# Autodesk Inventor assembly: robhand1
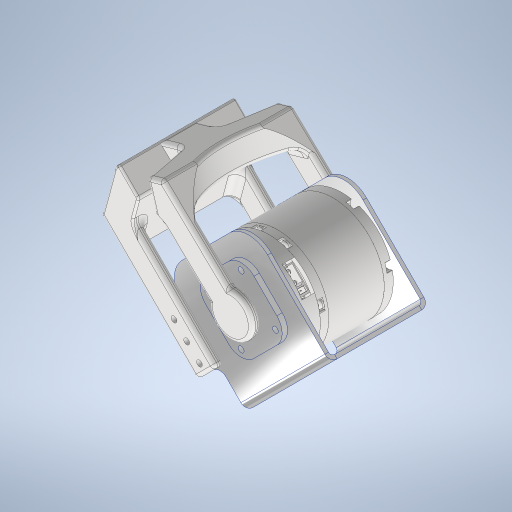
[picture p0: Inventor's stored thumbnail of the model, 512x512]
Saved by Autodesk Inventor 2024 (Build 280153000, 153)
## iProperties
Created: 2025-02-19
Part Number: robhand1
Document SubType Name: Assembly
Designer: tanoue_kota
Author: tanoue_kota
## Documents named in this file (7)
- C:\Users\田之上巧太\Documents\Inventor\RobArm\rob_hand1\robhand1.iam
- C:\Users\田之上巧太\Documents\Inventor\RobArm\Actuator\RS00\RS00.iam
- C:\Users\田之上巧太\Documents\Inventor\RobArm\rob_hand1\hand1_plate1.ipt
- C:\Users\田之上巧太\Documents\Inventor\RobArm\rob_hand1\hand1_part1.ipt
- C:\Users\田之上巧太\Documents\Inventor\RobArm\rob_hand1\hand1_part2.ipt
- C:\Users\田之上巧太\Documents\Inventor\RobArm\rob_hand1\hand1_part3.ipt
- C:\Users\田之上巧太\Documents\Inventor\RobArm\BasicParts\Bearing\NMB_LF1480ZZ\LF-1480ZZ.iam
## Components (6 placed, 6 different names)
1. RS00:1 [sub-assembly] — 回転:1, 回転:2, 回転:3, 回転:4, メイト:1, メイト:2
2. hand1_plate1:1 — 回転:1, 回転:2, 回転:5, 回転:6, 回転:7, 回転:8
3. hand1_part1:1 — 回転:3, 回転:4, メイト:1, メイト:2, メイト:3, メイト:4
4. hand1_part2:1 — 回転:5, 回転:6
5. hand1_part3:1 — 回転:7, 回転:8
6. LF-1480ZZ:1 [sub-assembly] — メイト:3, メイト:4
## Relationships (12: RevoluteJoint 8, Mate 4)
- 回転:1 [RevoluteJoint]: RS00:1 ↔ hand1_plate1:1
- 回転:2 [RevoluteJoint]: RS00:1 ↔ hand1_plate1:1
- 回転:3 [RevoluteJoint]: RS00:1 ↔ hand1_part1:1
- 回転:4 [RevoluteJoint]: RS00:1 ↔ hand1_part1:1
- メイト:1 [Mate]: RS00:1 ↔ hand1_part1:1
- メイト:2 [Mate]: RS00:1 ↔ hand1_part1:1
- 回転:5 [RevoluteJoint]: hand1_plate1:1 ↔ hand1_part2:1
- 回転:6 [RevoluteJoint]: hand1_plate1:1 ↔ hand1_part2:1
- 回転:7 [RevoluteJoint]: hand1_plate1:1 ↔ hand1_part3:1
- 回転:8 [RevoluteJoint]: hand1_plate1:1 ↔ hand1_part3:1
- メイト:3 [Mate]: hand1_part1:1 ↔ LF-1480ZZ:1
- メイト:4 [Mate]: hand1_part1:1 ↔ LF-1480ZZ:1
